# Autodesk Inventor assembly: wheelbasketback
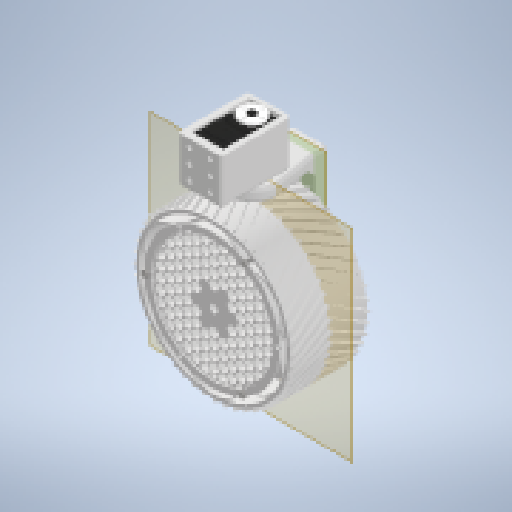
[picture p0: Inventor's stored thumbnail of the model, 512x512]
Saved by Autodesk Inventor 2025.3 (Build 293356000, 356)
## iProperties
Created: 2026-04-12
Part Number: wheelbasketback
Document SubType Name: Assembly
Designer: ksawe
Author: ksawe
## Documents named in this file (3)
- C:\Users\ksawe\OneDrive\Pulpit\Exomy v1\wersja2\wheelbasketback.iam
- C:\Users\ksawe\OneDrive\Pulpit\Exomy v1\wersja2\basketservoback.iam
- C:\Users\ksawe\OneDrive\Pulpit\Exomy v1\wersja2\kolowahacz.iam
## Components (2 placed, 2 different names)
1. basketservoback:1 [sub-assembly] — Mate:1, Mate:2, Mate:3
2. kolowahacz:2 [sub-assembly] — Mate:1, Mate:2, Mate:3
## Relationships (3: Mate 3)
- Mate:1: basketservoback:1 ↔ kolowahacz:2
- Mate:2: basketservoback:1 ↔ kolowahacz:2
- Mate:3: basketservoback:1 ↔ kolowahacz:2
